# Autodesk Inventor assembly: [Back] CoreXY <1>
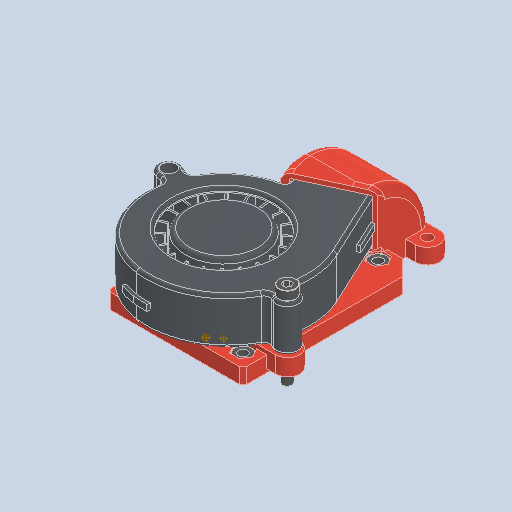
[picture p0: Inventor's stored thumbnail of the model, 512x512]
Saved by Autodesk Inventor 2022 (Build 260153000, 153)
## iProperties
Created: 2021-10-06
Part Number: [Back] CoreXY <1>
Document SubType Name: Assembly
Designer: Administrator
Title: [Back] CoreXY <1>
Author: Administrator
## Documents named in this file (5)
- Y:\Projects\Bibble0\Modified EVA Carriage\[Back] CoreXY _1_.iam
- Y:\Projects\Bibble0\Electronics\5015 fan.ipt
- Y:\Projects\Bibble0\Hardware\M3 x 25 mm  SHCS.ipt
- Y:\Projects\Bibble0\Modified EVA Carriage\back_corexy.ipt
- Y:\Projects\Bibble0\Hardware\M3 Hex Nut.ipt
## Components (10 placed, 4 different names)
1. 5015 fan:1 — Insert:1
2. DIN 912 M3 25 mm:1 — Insert:1
3. back_corexy:1
4. M3  Hex nut :3
5. M3  Hex nut :4
6. M3  Hex nut :5
7. M3  Hex nut :6
8. M3  Hex nut :7
9. M3  Hex nut :8
10. M3  Hex nut :9
## Relationships (1: Insert 1)
- Insert:1: 5015 fan:1 ↔ DIN 912 M3 25 mm:1
